# Autodesk Inventor assembly: FinalRev2
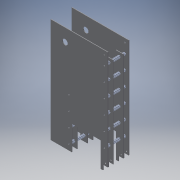
[picture p0: Inventor's stored thumbnail of the model, 180x180]
Saved by Autodesk Inventor 2016 (Build 200138000, 138)
## iProperties
Created: 2017-01-26
Part Number: FinalRev2
Document SubType Name: Assembly
Designer: Nick
Author: Nick
## Documents named in this file (5)
- C:\Users\madsenn\Documents\GitHub\Robot2017\Assemblies\FinalRev2.iam
- C:\Users\madsenn\Documents\GitHub\Robot2017\LauncherSidePlateRev2.ipt
- C:\Users\madsenn\Documents\GitHub\Robot2017\GearboxPlateRev3.ipt
- C:\Users\madsenn\Documents\GitHub\Robot2017\Parts\1InchChurro.ipt
- C:\Users\madsenn\Documents\GitHub\Robot2017\Parts\2InchChurro.ipt
## Components (34 placed, 4 different names)
1. LauncherSidePlateRev2:1 — Mate:28, Flush:1, Flush:2, Flush:3, Flush:4, Mate:30, Mate:32, Mate:35, Mate:48, Mate:50, Mate:53, Mate:66, Mate:70, Mate:74, Mate:124, Mate:125, Mate:126, Mate:127, Mate:128, Mate:129, Mate:130, Mate:131, Mate:132, Mate:133, Mate:134, Mate:135, Mate:136
2. LauncherSidePlateRev2:2 — Flush:1, Flush:4, Mate:30, Mate:75, Mate:76, Mate:77, Mate:78, Mate:79, Mate:80, Mate:81, Mate:82, Mate:83, Mate:84, Mate:85, Mate:86, Mate:89, Mate:90, Mate:91, Mate:92, Mate:93, Mate:94, Mate:95, Mate:96, Flush:5, Flush:6, Mate:97
3. GearboxPlateRev3:1 — Flush:5, Flush:6, Mate:97
4. GearboxPlateRev3:2 — Mate:27, Flush:2, Flush:3, Mate:31, Mate:33, Mate:49, Mate:51, Mate:52, Mate:54, Mate:55, Mate:67, Mate:68, Mate:69, Mate:72, Mate:73, Flush:7
5. 1InchChurro:1 — Mate:27, Mate:28, Mate:31, Mate:32
6. 1InchChurro:2 — Mate:33, Mate:35
7. 1InchChurro:3 — Mate:52, Mate:53
8. 1InchChurro:4 — Mate:54, Mate:55
9. 1InchChurro:5 — Mate:48, Mate:49
10. 1InchChurro:6 — Mate:50, Mate:51
11. 1InchChurro:9 — Mate:70, Mate:72
12. 1InchChurro:10 — Mate:68, Mate:69
13. 1InchChurro:11 — Mate:66, Mate:67
14. 1InchChurro:12 — Mate:73, Mate:74
15. 1InchChurro:13 — Mate:75, Mate:78
16. 1InchChurro:14 — Mate:76, Mate:77
17. 1InchChurro:15 — Mate:79, Mate:80
18. 1InchChurro:16 — Mate:81, Mate:83
19. 1InchChurro:17 — Mate:82, Mate:84
20. 1InchChurro:18 — Mate:85, Mate:86
21. 1InchChurro:20 — Mate:91, Mate:96
22. 1InchChurro:21 — Mate:89, Mate:90
23. 1InchChurro:22 — Mate:92, Mate:95
24. 1InchChurro:23 — Mate:93, Mate:94
25. 2InchChurro:1 — Mate:124
26. 2InchChurro:2 — Mate:125
27. 2InchChurro:3 — Mate:126
28. 2InchChurro:4 — Mate:127
29. 2InchChurro:5 — Mate:128
30. 2InchChurro:6 — Mate:129
31. 2InchChurro:7 — Mate:130
32. 2InchChurro:8 — Mate:131, Mate:135
33. 2InchChurro:9 — Mate:133, Mate:134
34. 2InchChurro:10 — Mate:132, Mate:136
## Relationships (64: Mate 57, Flush 7)
- Mate:27: GearboxPlateRev3:2 ↔ 1InchChurro:1
- Mate:28: LauncherSidePlateRev2:1 ↔ 1InchChurro:1
- Flush:1: LauncherSidePlateRev2:1 ↔ LauncherSidePlateRev2:2
- Flush:2: LauncherSidePlateRev2:1 ↔ GearboxPlateRev3:2
- Flush:3: LauncherSidePlateRev2:1 ↔ GearboxPlateRev3:2
- Flush:4: LauncherSidePlateRev2:1 ↔ LauncherSidePlateRev2:2
- Mate:30 (50.8 mm): LauncherSidePlateRev2:1 ↔ LauncherSidePlateRev2:2
- Mate:31: GearboxPlateRev3:2 ↔ 1InchChurro:1
- Mate:32: LauncherSidePlateRev2:1 ↔ 1InchChurro:1
- Mate:33: GearboxPlateRev3:2 ↔ 1InchChurro:2
- Mate:35: LauncherSidePlateRev2:1 ↔ 1InchChurro:2
- Mate:48: LauncherSidePlateRev2:1 ↔ 1InchChurro:5
- Mate:49: GearboxPlateRev3:2 ↔ 1InchChurro:5
- Mate:50: LauncherSidePlateRev2:1 ↔ 1InchChurro:6
- Mate:51: GearboxPlateRev3:2 ↔ 1InchChurro:6
- Mate:52: GearboxPlateRev3:2 ↔ 1InchChurro:3
- Mate:53: LauncherSidePlateRev2:1 ↔ 1InchChurro:3
- Mate:54: GearboxPlateRev3:2 ↔ 1InchChurro:4
- Mate:55: GearboxPlateRev3:2 ↔ 1InchChurro:4
- Mate:66: LauncherSidePlateRev2:1 ↔ 1InchChurro:11
- Mate:67: GearboxPlateRev3:2 ↔ 1InchChurro:11
- Mate:68: GearboxPlateRev3:2 ↔ 1InchChurro:10
- Mate:69: GearboxPlateRev3:2 ↔ 1InchChurro:10
- Mate:70: LauncherSidePlateRev2:1 ↔ 1InchChurro:9
- Mate:72: GearboxPlateRev3:2 ↔ 1InchChurro:9
- Mate:73: GearboxPlateRev3:2 ↔ 1InchChurro:12
- Mate:74: LauncherSidePlateRev2:1 ↔ 1InchChurro:12
- Mate:75: LauncherSidePlateRev2:2 ↔ 1InchChurro:13
- Mate:76: LauncherSidePlateRev2:2 ↔ 1InchChurro:14
- Mate:77: LauncherSidePlateRev2:2 ↔ 1InchChurro:14
- Mate:78: LauncherSidePlateRev2:2 ↔ 1InchChurro:13
- Mate:79: LauncherSidePlateRev2:2 ↔ 1InchChurro:15
- Mate:80: LauncherSidePlateRev2:2 ↔ 1InchChurro:15
- Mate:81: LauncherSidePlateRev2:2 ↔ 1InchChurro:16
- Mate:82: LauncherSidePlateRev2:2 ↔ 1InchChurro:17
- Mate:83: LauncherSidePlateRev2:2 ↔ 1InchChurro:16
- Mate:84: LauncherSidePlateRev2:2 ↔ 1InchChurro:17
- Mate:85: LauncherSidePlateRev2:2 ↔ 1InchChurro:18
- Mate:86: LauncherSidePlateRev2:2 ↔ 1InchChurro:18
- Mate:89: LauncherSidePlateRev2:2 ↔ 1InchChurro:21
- Mate:90: LauncherSidePlateRev2:2 ↔ 1InchChurro:21
- Mate:91: LauncherSidePlateRev2:2 ↔ 1InchChurro:20
- Mate:92: LauncherSidePlateRev2:2 ↔ 1InchChurro:22
- Mate:93: LauncherSidePlateRev2:2 ↔ 1InchChurro:23
- Mate:94: LauncherSidePlateRev2:2 ↔ 1InchChurro:23
- Mate:95: LauncherSidePlateRev2:2 ↔ 1InchChurro:22
- Mate:96: LauncherSidePlateRev2:2 ↔ 1InchChurro:20
- Flush:5: LauncherSidePlateRev2:2 ↔ GearboxPlateRev3:1
- Flush:6: LauncherSidePlateRev2:2 ↔ GearboxPlateRev3:1
- Mate:97 (25.4 mm): LauncherSidePlateRev2:2 ↔ GearboxPlateRev3:1
- Flush:7: GearboxPlateRev3:2
- Mate:124: LauncherSidePlateRev2:1 ↔ 2InchChurro:1
- Mate:125: LauncherSidePlateRev2:1 ↔ 2InchChurro:2
- Mate:126: LauncherSidePlateRev2:1 ↔ 2InchChurro:3
- Mate:127: LauncherSidePlateRev2:1 ↔ 2InchChurro:4
- Mate:128: LauncherSidePlateRev2:1 ↔ 2InchChurro:5
- Mate:129: LauncherSidePlateRev2:1 ↔ 2InchChurro:6
- Mate:130: LauncherSidePlateRev2:1 ↔ 2InchChurro:7
- Mate:131: LauncherSidePlateRev2:1 ↔ 2InchChurro:8
- Mate:132: LauncherSidePlateRev2:1 ↔ 2InchChurro:10
- Mate:133: LauncherSidePlateRev2:1 ↔ 2InchChurro:9
- Mate:134: LauncherSidePlateRev2:1 ↔ 2InchChurro:9
- Mate:135: LauncherSidePlateRev2:1 ↔ 2InchChurro:8
- Mate:136: LauncherSidePlateRev2:1 ↔ 2InchChurro:10
